# Autodesk Inventor assembly: 208
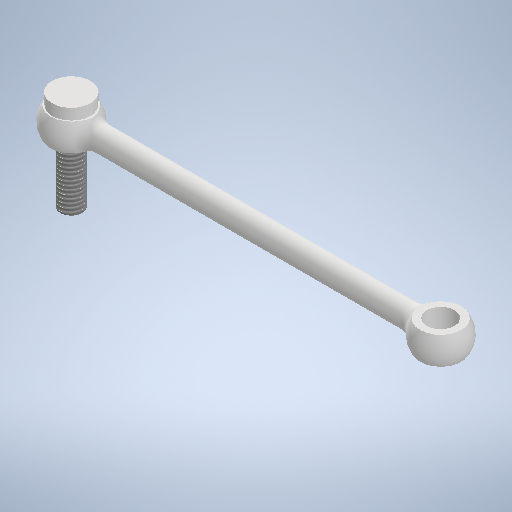
[picture p0: Inventor's stored thumbnail of the model, 512x512]
Saved by Autodesk Inventor 2025.1 (Build 291241000, 241)
## iProperties
Created: 2024-06-10
Part Number: 208
Document SubType Name: Assembly
Designer: ffogue
Author: ffogue
## Documents named in this file (3)
- C:\Users\ffogue\Downloads\Meine Projket\Paddle\208.iam
- C:\Users\ffogue\Downloads\Meine Projket\Paddle\2081.ipt
- C:\Users\ffogue\Downloads\Meine Projket\Paddle\2082.ipt
## Components (2 placed, 2 different names)
1. 2081:1 — Insert:2
2. 2082:2 — Insert:2
## Relationships (1: Insert 1)
- Insert:2: 2081:1 ↔ 2082:2
